# Autodesk Inventor assembly: Idler Sprocket
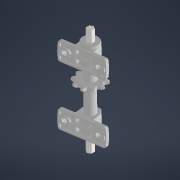
[picture p0: Inventor's stored thumbnail of the model, 180x180]
Saved by Autodesk Inventor 2022 (Build 260153000, 153)
## iProperties
Created: 2021-12-04
Part Number: Idler Sprocket
Document SubType Name: Assembly
Designer: izack
Author: izack
## Documents named in this file (8)
- D:\Robotics\ComputerAidedDesign\2021-22\FTC\#12456 Big Red\Drivetrain\Omni Wheel Drive\Idler Sprocket.iam
- D:\Robotics\ComputerAidedDesign\2021-22\FTC\Parts\REV Parts\10 Tooth #25 Sprocket - 4 Pack.ipt
- D:\Robotics\ComputerAidedDesign\2021-22\FTC\Parts\REV Parts\Through Bore Bearing - Long - 12 Pack.ipt
- D:\Robotics\ComputerAidedDesign\2021-22\FTC\Parts\REV Parts\5mm x 90mm Hex Shaft - 4 Pack.ipt
- D:\Robotics\ComputerAidedDesign\2021-22\FTC\Parts\REV Parts\15mm Spacer - 12 Pack.ipt
- D:\Robotics\ComputerAidedDesign\2021-22\FTC\Parts\REV Parts\3mm Spacer - 16 Pack.ipt
- D:\Robotics\ComputerAidedDesign\2021-22\FTC\Parts\REV Parts\1.5mm Spacers - 28 Pack.ipt
- D:\Robotics\ComputerAidedDesign\2021-22\FTC\Parts\REV Parts\15mm Bearing Pillow Block - 8 Pack.ipt
## Components (13 placed, 7 different names)
1. 10 Tooth #25 Sprocket - 4 Pack:1 — Mate:10, Mate:11, Mate:12
2. Through Bore Bearing - Long - 12 Pack:2 — Mate:1, Mate:2, Mate:3, Mate:7, Mate:9, Mate:20
3. 5mm x 90mm Hex Shaft - 4 Pack:1 — Mate:1, Mate:2, Mate:4, Mate:5, Mate:10, Mate:11, Flush:2
4. 15mm Spacer - 12 Pack:1 — Mate:22, Mate:23, Mate:24, Mate:25
5. 3mm Spacer - 16 Pack:1 — Mate:13, Mate:19, Mate:20, Mate:21
6. 1.5mm Spacers - 28 Pack:1 — Mate:16, Mate:17
7. 15mm Bearing Pillow Block - 8 Pack:1 — Mate:7, Mate:9, Flush:1, Mate:12, Mate:21
8. 15mm Bearing Pillow Block - 8 Pack:2 — Mate:6, Mate:8, Flush:1, Mate:25
9. Through Bore Bearing - Long - 12 Pack:3 — Mate:3, Mate:4, Mate:5, Mate:6, Mate:8, Flush:2, Mate:22
10. 3mm Spacer - 16 Pack:2 — Mate:13, Mate:14, Mate:15, Mate:18, Mate:19
11. 3mm Spacer - 16 Pack:3 — Mate:14, Mate:15, Mate:16, Mate:17, Mate:18
12. 3mm Spacer - 16 Pack:4 — Mate:23, Mate:24, Mate:26, Mate:27
13. 3mm Spacer - 16 Pack:5 — Mate:26, Mate:27
## Relationships (29: Mate 27, Flush 2)
- Mate:1: Through Bore Bearing - Long - 12 Pack:2 ↔ 5mm x 90mm Hex Shaft - 4 Pack:1
- Mate:2: Through Bore Bearing - Long - 12 Pack:2 ↔ 5mm x 90mm Hex Shaft - 4 Pack:1
- Mate:3 (64.4 mm): Through Bore Bearing - Long - 12 Pack:2 ↔ Through Bore Bearing - Long - 12 Pack:3
- Mate:4: 5mm x 90mm Hex Shaft - 4 Pack:1 ↔ Through Bore Bearing - Long - 12 Pack:3
- Mate:5: 5mm x 90mm Hex Shaft - 4 Pack:1 ↔ Through Bore Bearing - Long - 12 Pack:3
- Mate:6: 15mm Bearing Pillow Block - 8 Pack:2 ↔ Through Bore Bearing - Long - 12 Pack:3
- Mate:7: Through Bore Bearing - Long - 12 Pack:2 ↔ 15mm Bearing Pillow Block - 8 Pack:1
- Mate:8: 15mm Bearing Pillow Block - 8 Pack:2 ↔ Through Bore Bearing - Long - 12 Pack:3
- Mate:9: Through Bore Bearing - Long - 12 Pack:2 ↔ 15mm Bearing Pillow Block - 8 Pack:1
- Flush:1: 15mm Bearing Pillow Block - 8 Pack:1 ↔ 15mm Bearing Pillow Block - 8 Pack:2
- Mate:10: 10 Tooth #25 Sprocket - 4 Pack:1 ↔ 5mm x 90mm Hex Shaft - 4 Pack:1
- Mate:11: 10 Tooth #25 Sprocket - 4 Pack:1 ↔ 5mm x 90mm Hex Shaft - 4 Pack:1
- Flush:2 (-12 mm): 5mm x 90mm Hex Shaft - 4 Pack:1 ↔ Through Bore Bearing - Long - 12 Pack:3
- Mate:12 (4.2 mm): 10 Tooth #25 Sprocket - 4 Pack:1 ↔ 15mm Bearing Pillow Block - 8 Pack:1
- Mate:13: 3mm Spacer - 16 Pack:1 ↔ 3mm Spacer - 16 Pack:2
- Mate:14: 3mm Spacer - 16 Pack:2 ↔ 3mm Spacer - 16 Pack:3
- Mate:15: 3mm Spacer - 16 Pack:2 ↔ 3mm Spacer - 16 Pack:3
- Mate:16: 1.5mm Spacers - 28 Pack:1 ↔ 3mm Spacer - 16 Pack:3
- Mate:17: 1.5mm Spacers - 28 Pack:1 ↔ 3mm Spacer - 16 Pack:3
- Mate:18: 3mm Spacer - 16 Pack:2 ↔ 3mm Spacer - 16 Pack:3
- Mate:19: 3mm Spacer - 16 Pack:1 ↔ 3mm Spacer - 16 Pack:2
- Mate:20: Through Bore Bearing - Long - 12 Pack:2 ↔ 3mm Spacer - 16 Pack:1
- Mate:21: 3mm Spacer - 16 Pack:1 ↔ 15mm Bearing Pillow Block - 8 Pack:1
- Mate:22: 15mm Spacer - 12 Pack:1 ↔ Through Bore Bearing - Long - 12 Pack:3
- Mate:23: 15mm Spacer - 12 Pack:1 ↔ 3mm Spacer - 16 Pack:4
- Mate:24: 15mm Spacer - 12 Pack:1 ↔ 3mm Spacer - 16 Pack:4
- Mate:25: 15mm Spacer - 12 Pack:1 ↔ 15mm Bearing Pillow Block - 8 Pack:2
- Mate:26: 3mm Spacer - 16 Pack:4 ↔ 3mm Spacer - 16 Pack:5
- Mate:27: 3mm Spacer - 16 Pack:4 ↔ 3mm Spacer - 16 Pack:5
